# Autodesk Inventor assembly: MOGO Support Crossbrace
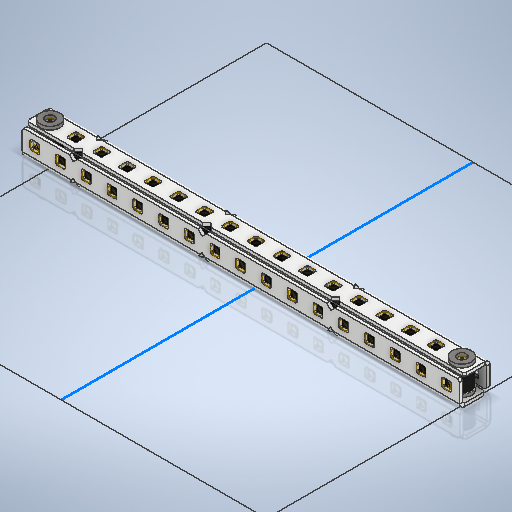
[picture p0: Inventor's stored thumbnail of the model, 512x512]
Saved by Autodesk Inventor 2026 (Build 300175000, 175)
## iProperties
Created: 2025-04-05
Part Number: MOGO Support Crossbrace
Document SubType Name: Assembly
Designer: avere
Author: avere
## Documents named in this file (6)
- C:\Users\avere\OneDrive\Documents\VEX-CAD\V5-CAD\Drivetrain\Braces\MOGO Support Crossbrace.iam
- C:\Users\avere\OneDrive\Documents\VEX-CAD\VEX-CAD-Inventor\Structure\Angle\Aluminum 1x1\Alu Angle 1x1x17.ipt
- C:\Users\avere\OneDrive\Documents\VEX-CAD\VEX-CAD-Inventor\Motion\Spacers\Spacer Nylon .375 OD\NSpacer .375 OD x .375.ipt
- C:\Users\avere\OneDrive\Documents\VEX-CAD\VEX-CAD-Inventor\Motion\Spacers\Spacer Nylon .375 OD.ipt
- C:\Users\avere\OneDrive\Documents\VEX-CAD\VEX-CAD-Inventor\Motion\Spacers\Washer Steel\SWasher .375 OD x .062500.ipt
- C:\Users\avere\OneDrive\Documents\VEX-CAD\VEX-CAD-Inventor\Motion\Spacers\Washer Steel.ipt
## Components (8 placed, 3 different names)
1. Alu Angle 1x1x17:1
2. Alu Angle 1x1x17:2 — Insert:6, Insert:7
3. NSpacer .375 OD x .375:1
4. SWasher .375 OD x .062500:1
5. NSpacer .375 OD x .375:2
6. SWasher .375 OD x .062500:2
7. SWasher .375 OD x .062500:3 — Insert:6
8. SWasher .375 OD x .062500:4 — Insert:7
## Relationships (8: Insert 7, Mate 1)
- [Insert] (11.1125 mm): Alu Angle 1x1x17:1 ↔ Alu Angle 1x1x17:2
- [Mate]: Alu Angle 1x1x17:1 ↔ Alu Angle 1x1x17:2
- [Insert]: NSpacer .375 OD x .375:1 ↔ SWasher .375 OD x .062500:1
- [Insert]: Alu Angle 1x1x17:1 ↔ SWasher .375 OD x .062500:1
- [Insert]: NSpacer .375 OD x .375:2 ↔ SWasher .375 OD x .062500:2
- [Insert]: Alu Angle 1x1x17:1 ↔ SWasher .375 OD x .062500:2
- Insert:6: Alu Angle 1x1x17:2 ↔ SWasher .375 OD x .062500:3
- Insert:7: Alu Angle 1x1x17:2 ↔ SWasher .375 OD x .062500:4
## Named parameters: d98_d96 = 0 mm
